# Autodesk Inventor assembly: mount
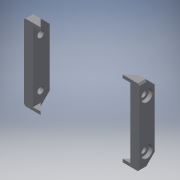
[picture p0: Inventor's stored thumbnail of the model, 180x180]
Saved by Autodesk Inventor 2016 (Build 200138000, 138)
## iProperties
Created: 2016-02-09
Part Number: mount
Document SubType Name: Assembly
Designer: element
Mass: 0.696141 g
Surface Area: 9.55276 cm^2
Volume: 0.696141 cm^3
Density: 1 g/cm^3
Author: element
## Documents named in this file (2)
- C:\Users\element\Desktop\technical_drawings\youbot\gripper\dynamixel_gripper\v2.0\inventor\motor_brackets\brackets.iam
- C:\Users\element\Desktop\technical_drawings\youbot\gripper\dynamixel_gripper\v2.0\inventor\motor_brackets\bracket.ipt
## Components (2 placed, 1 different names)
1. bracket:1 — Mate:1, Flush:1, Flush:2
2. bracket:2 — Mate:2, Mate:3, Mate:4
## Relationships (6: Mate 4, Flush 2)
- Mate:1: bracket:1
- Flush:1 (16 mm): bracket:1
- Flush:2: bracket:1
- Mate:2: bracket:2
- Mate:3: bracket:2
- Mate:4 (16 mm): bracket:2
